# Autodesk Inventor assembly: Sprung Button Assm DigiKey EG5980-ND
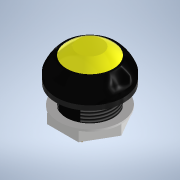
[picture p0: Inventor's stored thumbnail of the model, 180x180]
Saved by Autodesk Inventor 2021 (Build 250183000, 183)
## iProperties
Created: 2020-07-20
Part Number: Sprung Button Assm DigiKey EG5980-ND
Document SubType Name: Assembly
Designer: jgray
Author: jgray
## Documents named in this file (5)
- M:\Printed Electronics\Gas Sensors\Prototypes\Prototype II -Cartridge Reader V3\Sprung Button Assm DigiKey EG5980-ND.iam
- M:\Printed Electronics\Gas Sensors\Prototypes\Prototype II -Cartridge Reader V3\Sprung Button AntiVib M12 Washer.ipt
- M:\Printed Electronics\Gas Sensors\Prototypes\Prototype II -Cartridge Reader V3\Sprung Button DigiKey EG9580-ND.ipt
- M:\Printed Electronics\Gas Sensors\Prototypes\Prototype II -Cartridge Reader V3\Sprung Button Nut M12x075.ipt
- M:\Printed Electronics\Gas Sensors\Prototypes\Prototype II -Cartridge Reader V3\Sprung Button Seal Washer.ipt
## Components (4 placed, 4 different names)
1. Sprung Button AntiVib M12 Washer:1 — Mate:3, Mate:5
2. Sprung Button DigiKey EG9580-ND:1 — Mate:1, Mate:2, Mate:3, Mate:4
3. Sprung Button Nut M12x075:1 — Mate:4, Mate:5
4. Sprung Button Seal Washer:1 — Mate:1, Mate:2
## Relationships (5: Mate 5)
- Mate:1: Sprung Button DigiKey EG9580-ND:1 ↔ Sprung Button Seal Washer:1
- Mate:2: Sprung Button DigiKey EG9580-ND:1 ↔ Sprung Button Seal Washer:1
- Mate:3: Sprung Button AntiVib M12 Washer:1 ↔ Sprung Button DigiKey EG9580-ND:1
- Mate:4: Sprung Button DigiKey EG9580-ND:1 ↔ Sprung Button Nut M12x075:1
- Mate:5: Sprung Button AntiVib M12 Washer:1 ↔ Sprung Button Nut M12x075:1
